# Autodesk Inventor assembly: PMax6
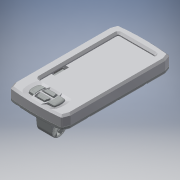
[picture p0: Inventor's stored thumbnail of the model, 180x180]
Saved by Autodesk Inventor 2018 (Build 220112000, 112)
## iProperties
Created: 2019-05-29
Part Number: PMax6
Document SubType Name: Assembly
Designer: Ash
Author: Ash
## Documents named in this file (7)
- C:\Autodesk\Skills 2019 Nationals\Competition\PMDay2\PMax6.iam
- C:\Autodesk\Skills 2019 Nationals\Competition\PMDay2\#2-KEYPAD.ipt
- C:\Autodesk\Skills 2019 Nationals\Competition\PMDay2\#4-GASKET(PMAX6).ipt
- C:\Autodesk\Skills 2019 Nationals\Competition\PMDay2\#5-BACK_COVER(PMAX6).ipt
- C:\Autodesk\Skills 2019 Nationals\Competition\PMDay1\Display_Plate2.ipt
- C:\Autodesk\Skills 2019 Nationals\Competition\PMDay1\Front_Cover2.ipt
- C:\Autodesk\Skills 2019 Nationals\Competition\PMDay2\#6-SCREW.ipt
## Components (15 placed, 6 different names)
1. #2-KEYPAD:1 — Mate:6, Mate:7, Mate:8, Mate:9, Mate:11
2. Display_Plate2:1 — Mate:7, Mate:10, Mate:11
3. Front_Cover2:1 — Mate:6, Mate:8, Mate:9, Mate:10, Mate:23, Mate:24, Mate:25
4. #5-BACK_COVER(PMAX6):1 — Mate:12, Mate:13, Mate:14, Mate:23, Mate:24, Mate:25, Mate:26, Mate:27, Mate:28, Mate:29, Mate:30, Mate:31, Mate:32, Mate:33, Mate:34, Mate:35, Mate:36
5. #4-GASKET(PMAX6):1 — Mate:12, Mate:13, Mate:14
6. #6-SCREW:1 — Mate:28, Flush:39, Flush:40
7. #6-SCREW:2 — Mate:27, Flush:38, Flush:39
8. #6-SCREW:3 — Mate:32, Flush:43, Flush:44
9. #6-SCREW:4 — Mate:31, Flush:42, Flush:43, Mate:36
10. #6-SCREW:5 — Mate:29, Flush:40, Flush:41
11. #6-SCREW:6 — Mate:33, Flush:44
12. #6-SCREW:7 — Mate:34, Flush:37, Flush:1
13. #6-SCREW:8 — Mate:35, Flush:37
14. #6-SCREW:9 — Mate:26, Flush:1, Flush:38
15. #6-SCREW:10 — Mate:30, Flush:41, Flush:42
## Relationships (32: Mate 23, Flush 9)
- Mate:6 (6.35 mm): #2-KEYPAD:1 ↔ Front_Cover2:1
- Mate:7: #2-KEYPAD:1 ↔ Display_Plate2:1
- Mate:8: #2-KEYPAD:1 ↔ Front_Cover2:1
- Mate:9 (46.7868 mm): #2-KEYPAD:1 ↔ Front_Cover2:1
- Mate:10: Display_Plate2:1 ↔ Front_Cover2:1
- Mate:11: #2-KEYPAD:1 ↔ Display_Plate2:1
- Mate:12: #5-BACK_COVER(PMAX6):1 ↔ #4-GASKET(PMAX6):1
- Mate:13: #5-BACK_COVER(PMAX6):1 ↔ #4-GASKET(PMAX6):1
- Mate:14: #5-BACK_COVER(PMAX6):1 ↔ #4-GASKET(PMAX6):1
- Mate:23: Front_Cover2:1 ↔ #5-BACK_COVER(PMAX6):1
- Mate:24: Front_Cover2:1 ↔ #5-BACK_COVER(PMAX6):1
- Mate:25: Front_Cover2:1 ↔ #5-BACK_COVER(PMAX6):1
- Mate:26: #5-BACK_COVER(PMAX6):1 ↔ #6-SCREW:9
- Mate:27: #5-BACK_COVER(PMAX6):1 ↔ #6-SCREW:2
- Mate:28: #5-BACK_COVER(PMAX6):1 ↔ #6-SCREW:1
- Mate:29: #5-BACK_COVER(PMAX6):1 ↔ #6-SCREW:5
- Mate:30: #5-BACK_COVER(PMAX6):1 ↔ #6-SCREW:10
- Mate:31: #5-BACK_COVER(PMAX6):1 ↔ #6-SCREW:4
- Mate:32: #5-BACK_COVER(PMAX6):1 ↔ #6-SCREW:3
- Mate:33: #5-BACK_COVER(PMAX6):1 ↔ #6-SCREW:6
- Mate:34: #5-BACK_COVER(PMAX6):1 ↔ #6-SCREW:7
- Mate:35: #5-BACK_COVER(PMAX6):1 ↔ #6-SCREW:8
- Flush:37: #6-SCREW:7 ↔ #6-SCREW:8
- Flush:1: #6-SCREW:7 ↔ #6-SCREW:9
- Flush:38: #6-SCREW:2 ↔ #6-SCREW:9
- Flush:39: #6-SCREW:1 ↔ #6-SCREW:2
- Flush:40: #6-SCREW:1 ↔ #6-SCREW:5
- Flush:41: #6-SCREW:5 ↔ #6-SCREW:10
- Flush:42: #6-SCREW:4 ↔ #6-SCREW:10
- Flush:43: #6-SCREW:3 ↔ #6-SCREW:4
- Flush:44: #6-SCREW:3 ↔ #6-SCREW:6
- Mate:36: #5-BACK_COVER(PMAX6):1 ↔ #6-SCREW:4
